# Autodesk Inventor assembly: RAI_Assembly
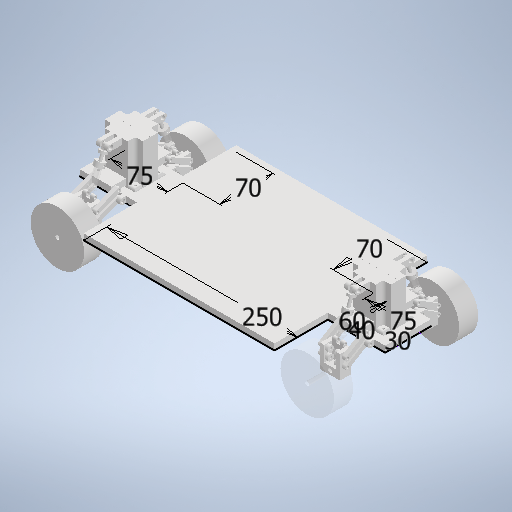
[picture p0: Inventor's stored thumbnail of the model, 512x512]
Saved by Autodesk Inventor 2025.2 (Build 292293000, 293)
## iProperties
Created: 2025-01-03
Part Number: RAI_Assembly
Document SubType Name: Assembly
Designer: SEON
Author: SEON
## Documents named in this file (8)
- C:\Users\SEON\Documents\Inventor\ProjectRAI\RAI_Assembly.iam
- C:\Users\SEON\Documents\Inventor\ProjectRAI\BottomFrame.ipt
- C:\Users\SEON\Documents\Inventor\ProjectRAI\SuspensionSupporter.ipt
- C:\Users\SEON\Documents\Inventor\ProjectRAI\TireDummy.ipt
- C:\Users\SEON\Documents\Inventor\ProjectRAI\SteeringFrame.ipt
- C:\Users\SEON\Documents\Inventor\ProjectRAI\SteeringConnector.ipt
- C:\Users\SEON\Documents\Inventor\ProjectRAI\SuspensionFrame.ipt
- C:\Users\SEON\Documents\Inventor\ProjectRAI\SuspensionAssembly.iam
## Components (49 placed, 7 different names)
1. BottomFrame:1 — 메이트:1, 메이트:2, 메이트:3, 메이트:5, 메이트:6, 메이트:17, 메이트:18, 메이트:21, 메이트:37, 메이트:43, 메이트:55, 메이트:62, 메이트:63, 메이트:64, 메이트:65, 메이트:67, 메이트:89, 메이트:91, 메이트:93, 메이트:111, 메이트:113, 메이트:115
2. SuspensionSupporter:1 — 메이트:1, 메이트:2, 메이트:3, 메이트:4, 메이트:46, 메이트:56, 메이트:58, 메이트:59
3. SuspensionSupporter:2 — 메이트:4, 메이트:5, 메이트:6, 메이트:23, 메이트:26, 메이트:35
4. TireDummy:1 — 메이트:7, 메이트:8
5. SteeringFrame:1 — 메이트:7, 메이트:8, 메이트:9, 메이트:10, 메이트:11, 메이트:12, 메이트:19, 메이트:24, 메이트:27, 메이트:28, 메이트:29, 메이트:30, 메이트:33, 메이트:34
6. SuspensionFrame:2 — 메이트:13, 메이트:14, 메이트:18, 메이트:21
7. SteeringConnector:3 — 메이트:9, 메이트:10, 메이트:13, 메이트:14
8. SteeringConnector:4 — 메이트:11, 메이트:12, 메이트:15, 메이트:16
9. SuspensionFrame:3 — 메이트:15, 메이트:16, 메이트:17
10. SuspensionFrame:4 — 메이트:19, 메이트:23, 메이트:31
11. SuspensionFrame:5 — 메이트:24, 메이트:26, 메이트:32
12. SteeringConnector:5 — 메이트:27, 메이트:28, 메이트:32
13. SteeringConnector:6 — 메이트:29, 메이트:30, 메이트:31
14. SuspensionAssembly:1 [sub-assembly] — 메이트:33, 메이트:34, 메이트:35
15. SuspensionFrame:6 — 메이트:44, 메이트:45, 메이트:46
16. SuspensionFrame:7 — 메이트:53, 메이트:54, 메이트:55
17. SuspensionFrame:8 — 메이트:36, 메이트:37, 메이트:42, 메이트:43
18. SuspensionFrame:9 — 메이트:51, 메이트:52, 메이트:56
19. SteeringFrame:2 — 메이트:36, 메이트:38, 메이트:39, 메이트:40, 메이트:41, 메이트:45, 메이트:47, 메이트:48, 메이트:49, 메이트:50, 메이트:57, 메이트:60, 메이트:61
20. SuspensionAssembly:2 [sub-assembly] — 메이트:57, 메이트:58, 메이트:59
21. SteeringConnector:7 — 메이트:48, 메이트:49, 메이트:51, 메이트:52
22. SteeringConnector:8 — 메이트:38, 메이트:39, 메이트:44
23. SteeringConnector:9 — 메이트:47, 메이트:50, 메이트:53, 메이트:54
24. SteeringConnector:10 — 메이트:40, 메이트:41, 메이트:42
25. TireDummy:2 — 메이트:60, 메이트:61
26. SuspensionSupporter:3 — 메이트:62, 메이트:66, 메이트:67, 메이트:68, 메이트:69, 메이트:90, 메이트:92
27. SuspensionSupporter:4 — 메이트:63, 메이트:64, 메이트:65, 메이트:66, 메이트:70, 메이트:71, 메이트:112, 메이트:114
28. SuspensionAssembly:3 [sub-assembly] — 메이트:68, 메이트:69, 메이트:88
29. SuspensionAssembly:4 [sub-assembly] — 메이트:70, 메이트:71, 메이트:116
30. SuspensionFrame:10 — 메이트:84, 메이트:85, 메이트:93
31. SuspensionFrame:11 — 메이트:82, 메이트:83, 메이트:90
32. SuspensionFrame:12 — 메이트:86, 메이트:87, 메이트:92
33. SuspensionFrame:13 — 메이트:80, 메이트:81, 메이트:89, 메이트:91
34. SteeringFrame:3 — 메이트:72, 메이트:73, 메이트:74, 메이트:75, 메이트:76, 메이트:77, 메이트:78, 메이트:79, 메이트:88, 메이트:118, 메이트:119
35. SteeringConnector:11 — 메이트:77, 메이트:79, 메이트:86, 메이트:87
36. SteeringConnector:12 — 메이트:76, 메이트:78, 메이트:84, 메이트:85
37. SteeringConnector:13 — 메이트:72, 메이트:74, 메이트:82, 메이트:83
38. SteeringConnector:14 — 메이트:73, 메이트:75, 메이트:80, 메이트:81
39. SuspensionFrame:14 — 메이트:113
40. SuspensionFrame:15 — 메이트:112
41. SuspensionFrame:16 — 메이트:114
42. SuspensionFrame:17 — 메이트:111, 메이트:115
43. SteeringFrame:4 — 메이트:116, 메이트:117, 메이트:120
44. SteeringConnector:15
45. SteeringConnector:16
46. SteeringConnector:17
47. SteeringConnector:18
48. TireDummy:3 — 메이트:117, 메이트:120
49. TireDummy:4 — 메이트:118, 메이트:119
## Relationships (116: Mate 116)
- 메이트:1 [Mate]: BottomFrame:1 ↔ SuspensionSupporter:1
- 메이트:2 [Mate]: BottomFrame:1 ↔ SuspensionSupporter:1
- 메이트:3 [Mate]: BottomFrame:1 ↔ SuspensionSupporter:1
- 메이트:4 [Mate]: SuspensionSupporter:1 ↔ SuspensionSupporter:2
- 메이트:5 [Mate]: BottomFrame:1 ↔ SuspensionSupporter:2
- 메이트:6 [Mate]: BottomFrame:1 ↔ SuspensionSupporter:2
- 메이트:7 [Mate]: TireDummy:1 ↔ SteeringFrame:1
- 메이트:8 [Mate] (5 mm): TireDummy:1 ↔ SteeringFrame:1
- 메이트:9 [Mate]: SteeringFrame:1 ↔ SteeringConnector:3
- 메이트:10 [Mate]: SteeringFrame:1 ↔ SteeringConnector:3
- 메이트:11 [Mate]: SteeringFrame:1 ↔ SteeringConnector:4
- 메이트:12 [Mate]: SteeringFrame:1 ↔ SteeringConnector:4
- 메이트:13 [Mate]: SuspensionFrame:2 ↔ SteeringConnector:3
- 메이트:14 [Mate]: SuspensionFrame:2 ↔ SteeringConnector:3
- 메이트:15 [Mate]: SteeringConnector:4 ↔ SuspensionFrame:3
- 메이트:16 [Mate]: SteeringConnector:4 ↔ SuspensionFrame:3
- 메이트:17 [Mate]: BottomFrame:1 ↔ SuspensionFrame:3
- 메이트:18 [Mate]: BottomFrame:1 ↔ SuspensionFrame:2
- 메이트:19 [Mate]: SteeringFrame:1 ↔ SuspensionFrame:4
- 메이트:21 [Mate]: BottomFrame:1 ↔ SuspensionFrame:2
- 메이트:23 [Mate]: SuspensionSupporter:2 ↔ SuspensionFrame:4
- 메이트:24 [Mate]: SteeringFrame:1 ↔ SuspensionFrame:5
- 메이트:26 [Mate]: SuspensionSupporter:2 ↔ SuspensionFrame:5
- 메이트:27 [Mate]: SteeringFrame:1 ↔ SteeringConnector:5
- 메이트:28 [Mate]: SteeringFrame:1 ↔ SteeringConnector:5
- 메이트:29 [Mate]: SteeringFrame:1 ↔ SteeringConnector:6
- 메이트:30 [Mate]: SteeringFrame:1 ↔ SteeringConnector:6
- 메이트:31 [Mate]: SuspensionFrame:4 ↔ SteeringConnector:6
- 메이트:32 [Mate]: SuspensionFrame:5 ↔ SteeringConnector:5
- 메이트:33 [Mate]: SteeringFrame:1 ↔ SuspensionAssembly:1
- 메이트:34 [Mate]: SteeringFrame:1 ↔ SuspensionAssembly:1
- 메이트:35 [Mate]: SuspensionSupporter:2 ↔ SuspensionAssembly:1
- 메이트:36 [Mate]: SuspensionFrame:8 ↔ SteeringFrame:2
- 메이트:37 [Mate]: BottomFrame:1 ↔ SuspensionFrame:8
- 메이트:38 [Mate]: SteeringFrame:2 ↔ SteeringConnector:8
- 메이트:39 [Mate]: SteeringFrame:2 ↔ SteeringConnector:8
- 메이트:40 [Mate]: SteeringFrame:2 ↔ SteeringConnector:10
- 메이트:41 [Mate]: SteeringFrame:2 ↔ SteeringConnector:10
- 메이트:42 [Mate]: SuspensionFrame:8 ↔ SteeringConnector:10
- 메이트:43 [Mate]: BottomFrame:1 ↔ SuspensionFrame:8
- 메이트:44 [Mate]: SuspensionFrame:6 ↔ SteeringConnector:8
- 메이트:45 [Mate]: SuspensionFrame:6 ↔ SteeringFrame:2
- 메이트:46 [Mate]: SuspensionSupporter:1 ↔ SuspensionFrame:6
- 메이트:47 [Mate]: SteeringFrame:2 ↔ SteeringConnector:9
- 메이트:48 [Mate]: SteeringFrame:2 ↔ SteeringConnector:7
- 메이트:49 [Mate]: SteeringFrame:2 ↔ SteeringConnector:7
- 메이트:50 [Mate]: SteeringFrame:2 ↔ SteeringConnector:9
- 메이트:51 [Mate]: SuspensionFrame:9 ↔ SteeringConnector:7
- 메이트:52 [Mate]: SuspensionFrame:9 ↔ SteeringConnector:7
- 메이트:53 [Mate]: SuspensionFrame:7 ↔ SteeringConnector:9
- 메이트:54 [Mate]: SuspensionFrame:7 ↔ SteeringConnector:9
- 메이트:55 [Mate]: BottomFrame:1 ↔ SuspensionFrame:7
- 메이트:56 [Mate]: SuspensionSupporter:1 ↔ SuspensionFrame:9
- 메이트:57 [Mate]: SteeringFrame:2 ↔ SuspensionAssembly:2
- 메이트:58 [Mate]: SuspensionSupporter:1 ↔ SuspensionAssembly:2
- 메이트:59 [Mate]: SuspensionSupporter:1 ↔ SuspensionAssembly:2
- 메이트:60 [Mate]: SteeringFrame:2 ↔ TireDummy:2
- 메이트:61 [Mate] (5 mm): SteeringFrame:2 ↔ TireDummy:2
- 메이트:62 [Mate]: BottomFrame:1 ↔ SuspensionSupporter:3
- 메이트:63 [Mate]: BottomFrame:1 ↔ SuspensionSupporter:4
- 메이트:64 [Mate]: BottomFrame:1 ↔ SuspensionSupporter:4
- 메이트:65 [Mate]: BottomFrame:1 ↔ SuspensionSupporter:4
- 메이트:66 [Mate]: SuspensionSupporter:3 ↔ SuspensionSupporter:4
- 메이트:67 [Mate]: BottomFrame:1 ↔ SuspensionSupporter:3
- 메이트:68 [Mate]: SuspensionSupporter:3 ↔ SuspensionAssembly:3
- 메이트:69 [Mate]: SuspensionSupporter:3 ↔ SuspensionAssembly:3
- 메이트:70 [Mate]: SuspensionSupporter:4 ↔ SuspensionAssembly:4
- 메이트:71 [Mate]: SuspensionSupporter:4 ↔ SuspensionAssembly:4
- 메이트:72 [Mate]: SteeringFrame:3 ↔ SteeringConnector:13
- 메이트:73 [Mate]: SteeringFrame:3 ↔ SteeringConnector:14
- 메이트:74 [Mate]: SteeringFrame:3 ↔ SteeringConnector:13
- 메이트:75 [Mate]: SteeringFrame:3 ↔ SteeringConnector:14
- 메이트:76 [Mate]: SteeringFrame:3 ↔ SteeringConnector:12
- 메이트:77 [Mate]: SteeringFrame:3 ↔ SteeringConnector:11
- 메이트:78 [Mate]: SteeringFrame:3 ↔ SteeringConnector:12
- 메이트:79 [Mate]: SteeringFrame:3 ↔ SteeringConnector:11
- 메이트:80 [Mate]: SuspensionFrame:13 ↔ SteeringConnector:14
- 메이트:81 [Mate]: SuspensionFrame:13 ↔ SteeringConnector:14
- 메이트:82 [Mate]: SuspensionFrame:11 ↔ SteeringConnector:13
- 메이트:83 [Mate]: SuspensionFrame:11 ↔ SteeringConnector:13
- 메이트:84 [Mate]: SuspensionFrame:10 ↔ SteeringConnector:12
- 메이트:85 [Mate]: SuspensionFrame:10 ↔ SteeringConnector:12
- 메이트:86 [Mate]: SuspensionFrame:12 ↔ SteeringConnector:11
- 메이트:87 [Mate]: SuspensionFrame:12 ↔ SteeringConnector:11
- 메이트:88 [Mate]: SuspensionAssembly:3 ↔ SteeringFrame:3
- 메이트:89 [Mate]: BottomFrame:1 ↔ SuspensionFrame:13
- 메이트:90 [Mate]: SuspensionSupporter:3 ↔ SuspensionFrame:11
- 메이트:91 [Mate]: BottomFrame:1 ↔ SuspensionFrame:13
- 메이트:92 [Mate]: SuspensionSupporter:3 ↔ SuspensionFrame:12
- 메이트:93 [Mate]: BottomFrame:1 ↔ SuspensionFrame:10
- [Mate]: SteeringFrame:4 ↔ SteeringConnector:17
- [Mate]: SteeringFrame:4 ↔ SteeringConnector:18
- [Mate]: SteeringFrame:4 ↔ SteeringConnector:17
- [Mate]: SteeringFrame:4 ↔ SteeringConnector:18
- [Mate]: SteeringFrame:4 ↔ SteeringConnector:16
- [Mate]: SteeringFrame:4 ↔ SteeringConnector:15
- [Mate]: SteeringFrame:4 ↔ SteeringConnector:16
- [Mate]: SteeringFrame:4 ↔ SteeringConnector:15
- [Mate]: SuspensionFrame:17 ↔ SteeringConnector:18
- [Mate]: SuspensionFrame:17 ↔ SteeringConnector:18
- [Mate]: SuspensionFrame:15 ↔ SteeringConnector:17
- [Mate]: SuspensionFrame:15 ↔ SteeringConnector:17
- [Mate]: SuspensionFrame:14 ↔ SteeringConnector:16
- [Mate]: SuspensionFrame:14 ↔ SteeringConnector:16
- [Mate]: SuspensionFrame:16 ↔ SteeringConnector:15
- [Mate]: SuspensionFrame:16 ↔ SteeringConnector:15
- 메이트:111 [Mate]: BottomFrame:1 ↔ SuspensionFrame:17
- 메이트:112 [Mate]: SuspensionSupporter:4 ↔ SuspensionFrame:15
- 메이트:113 [Mate]: BottomFrame:1 ↔ SuspensionFrame:14
- 메이트:114 [Mate]: SuspensionSupporter:4 ↔ SuspensionFrame:16
- 메이트:115 [Mate]: BottomFrame:1 ↔ SuspensionFrame:17
- 메이트:116 [Mate]: SuspensionAssembly:4 ↔ SteeringFrame:4
- 메이트:117 [Mate]: SteeringFrame:4 ↔ TireDummy:3
- 메이트:118 [Mate]: SteeringFrame:3 ↔ TireDummy:4
- 메이트:119 [Mate] (5 mm): SteeringFrame:3 ↔ TireDummy:4
- 메이트:120 [Mate] (5 mm): SteeringFrame:4 ↔ TireDummy:3
## Named parameters: d98_d82 = 0 mm, d99_d83 = 0 mm, d100_d84 = 0 mm, d101_d85 = 0 mm, d102_d86 = 0 mm, d103_d87 = 0 mm, d104_d88 = 0 mm, d105_d89 = 0 mm, d106_d90 = 0 mm, d107_d91 = 0 mm, d109_d76 = 0 mm, d110_d77 = 0 mm, d111_d78 = 0 mm, d112_d79 = 0 mm, d113_d80 = 0 mm, d114_d81 = 0 mm
